# Autodesk Inventor assembly: AL-250G Lathe Assembly (Stock)
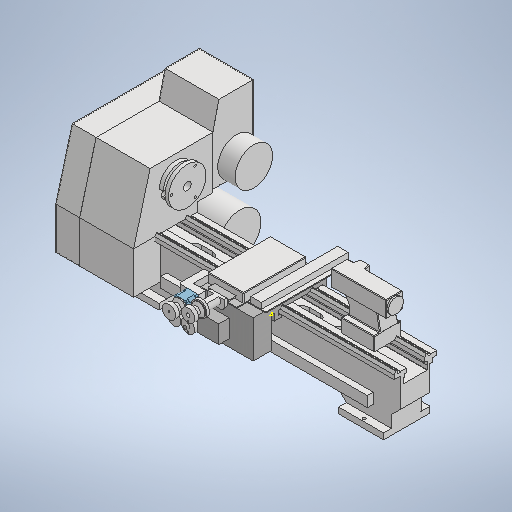
[picture p0: Inventor's stored thumbnail of the model, 512x512]
Saved by Autodesk Inventor 2025.1 (Build 291241000, 241)
## iProperties
Created: 2024-08-21
Part Number: AL-250G Lathe Assembly (Stock)
Document SubType Name: Assembly
Designer: max_d
Author: max_d
## Documents named in this file (15)
- E:\00 Network Folder\1. Projects\P0. Digital Twins - OTS Parts - Environment Models\Machine Shed\Shed CAD Files\AL-250G Lathe Assembly (Stock).iam
- E:\00 Network Folder\1. Projects\P0. Digital Twins - OTS Parts - Environment Models\Machine Shed\Shed CAD Files\AL-250G Geared Head Lathe.ipt
- E:\00 Network Folder\1. Projects\P0. Digital Twins - OTS Parts - Environment Models\Machine Shed\Shed CAD Files\Chuck Backplate.ipt
- E:\00 Network Folder\1. Projects\P0. Digital Twins - OTS Parts - Environment Models\Machine Shed\Shed CAD Files\Sanou K11-125 3-Jaw Chuck.ipt
- E:\00 Network Folder\1. Projects\P0. Digital Twins - OTS Parts - Environment Models\Machine Shed\Shed CAD Files\Tail Stock.ipt
- E:\00 Network Folder\1. Projects\P0. Digital Twins - OTS Parts - Environment Models\Machine Shed\Shed CAD Files\Apron.ipt
- E:\00 Network Folder\1. Projects\P0. Digital Twins - OTS Parts - Environment Models\Machine Shed\Shed CAD Files\LinearScale-690mm.ipt
- E:\00 Network Folder\1. Projects\P0. Digital Twins - OTS Parts - Environment Models\Machine Shed\Shed CAD Files\XaxisScaleMount.ipt
- E:\00 Network Folder\1. Projects\P0. Digital Twins - OTS Parts - Environment Models\Machine Shed\Shed CAD Files\LinearScale-290mm.ipt
- E:\00 Network Folder\1. Projects\P0. Digital Twins - OTS Parts - Environment Models\Machine Shed\Shed CAD Files\Cross Slide.ipt
- E:\00 Network Folder\1. Projects\P0. Digital Twins - OTS Parts - Environment Models\Machine Shed\Shed CAD Files\Vbelt Drive Pulley.ipt
- E:\00 Network Folder\1. Projects\P0. Digital Twins - OTS Parts - Environment Models\Machine Shed\Nema17 Stepper Motor\Nema17.ipt
- E:\00 Network Folder\1. Projects\P0. Digital Twins - OTS Parts - Environment Models\Machine Shed\Shed CAD Files\Vbelt Slave Pulley.ipt
- E:\00 Network Folder\1. Projects\P0. Digital Twins - OTS Parts - Environment Models\Machine Shed\Shed CAD Files\ZaxisMotorMount.ipt
- E:\00 Network Folder\1. Projects\P0. Digital Twins - OTS Parts - Environment Models\Machine Shed\Shed CAD Files\XaxisMotorMount.ipt
## Components (17 placed, 14 different names)
1. AL-250G Geared Head Lathe:1 — Mate:1, Mate:2, Mate:4, Mate:5, Mate:6, Mate:7, Mate:8, Flush:1, Mate:9
2. Chuck Backplate:1 — Mate:1, Mate:2, Mate:3
3. Sanou K11-125 3-Jaw Chuck:1 — Mate:3
4. Tail Stock:1 — Mate:4, Mate:5
5. Apron:1 — Mate:6, Mate:7, Mate:10, Mate:11, Flush:2, Mate:13, Mate:14, Flush:20, Flush:5, Mate:20, Flush:6, Flush:7, Flush:8, Mate:21, Mate:22, Mate:25, Mate:26, Mate:29, Flush:21, Mate:31, Mate:32
6. LinearScale-690mm:1 — Mate:8, Flush:1, Mate:9
7. XaxisScaleMount:1 — Mate:10, Mate:11, Flush:2, Mate:12, Flush:3, Flush:4
8. LinearScale-290mm:1 — Mate:12, Flush:3, Flush:4
9. Cross Slide:1 — Mate:13, Mate:14
10. Vbelt Drive Pulley:1 — Mate:24, Mate:27
11. Vbelt Drive Pulley:2 — Mate:23, Mate:28
12. Nema17:1 — Flush:20, Flush:6, Flush:7, Mate:24, Mate:27, Flush:22
13. Nema17:2 — Flush:5, Mate:20, Flush:8, Mate:23, Mate:28, Mate:30
14. Vbelt Slave Pulley:1 — Mate:21, Mate:26
15. Vbelt Slave Pulley:2 — Mate:22, Mate:25
16. ZaxisMotorMount:1 — Mate:29, Flush:21, Mate:30
17. XaxisMotorMount:1 — Mate:31, Mate:32, Flush:22
## Relationships (38: Mate 27, Flush 11)
- Mate:1: AL-250G Geared Head Lathe:1 ↔ Chuck Backplate:1
- Mate:2: AL-250G Geared Head Lathe:1 ↔ Chuck Backplate:1
- Mate:3: Chuck Backplate:1 ↔ Sanou K11-125 3-Jaw Chuck:1
- Mate:4: AL-250G Geared Head Lathe:1 ↔ Tail Stock:1
- Mate:5: AL-250G Geared Head Lathe:1 ↔ Tail Stock:1
- Mate:6: AL-250G Geared Head Lathe:1 ↔ Apron:1
- Mate:7: AL-250G Geared Head Lathe:1 ↔ Apron:1
- Mate:8: AL-250G Geared Head Lathe:1 ↔ LinearScale-690mm:1
- Flush:1: AL-250G Geared Head Lathe:1 ↔ LinearScale-690mm:1
- Mate:9 (20 mm): AL-250G Geared Head Lathe:1 ↔ LinearScale-690mm:1
- Mate:10: Apron:1 ↔ XaxisScaleMount:1
- Mate:11 (2 mm): Apron:1 ↔ XaxisScaleMount:1
- Flush:2 (35 mm): Apron:1 ↔ XaxisScaleMount:1
- Mate:12: XaxisScaleMount:1 ↔ LinearScale-290mm:1
- Flush:3 (10 mm): XaxisScaleMount:1 ↔ LinearScale-290mm:1
- Flush:4: XaxisScaleMount:1 ↔ LinearScale-290mm:1
- Mate:13: Apron:1 ↔ Cross Slide:1
- Mate:14: Apron:1 ↔ Cross Slide:1
- Flush:20: Apron:1 ↔ Nema17:1
- Flush:5: Apron:1 ↔ Nema17:2
- Mate:20: Apron:1 ↔ Nema17:2
- Flush:6: Apron:1 ↔ Nema17:1
- Flush:7: Apron:1 ↔ Nema17:1
- Flush:8 (14 mm): Apron:1 ↔ Nema17:2
- Mate:21: Apron:1 ↔ Vbelt Slave Pulley:1
- Mate:22: Apron:1 ↔ Vbelt Slave Pulley:2
- Mate:23: Vbelt Drive Pulley:2 ↔ Nema17:2
- Mate:24: Vbelt Drive Pulley:1 ↔ Nema17:1
- Mate:25: Apron:1 ↔ Vbelt Slave Pulley:2
- Mate:26: Apron:1 ↔ Vbelt Slave Pulley:1
- Mate:27: Vbelt Drive Pulley:1 ↔ Nema17:1
- Mate:28: Vbelt Drive Pulley:2 ↔ Nema17:2
- Mate:29: Apron:1 ↔ ZaxisMotorMount:1
- Flush:21: Apron:1 ↔ ZaxisMotorMount:1
- Mate:30: Nema17:2 ↔ ZaxisMotorMount:1
- Mate:31: Apron:1 ↔ XaxisMotorMount:1
- Mate:32: Apron:1 ↔ XaxisMotorMount:1
- Flush:22: Nema17:1 ↔ XaxisMotorMount:1
